# Autodesk Inventor assembly: Jersey_FEA_assembly
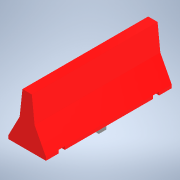
[picture p0: Inventor's stored thumbnail of the model, 180x180]
Saved by Autodesk Inventor 2022 (Build 260153000, 153)
## iProperties
Created: 2021-11-09
Part Number: Jersey_FEA_assembly
Document SubType Name: Assembly
Designer: kibandi
Author: kibandi
## Documents named in this file (3)
- C:\academics\YEAR 4\4.2\DOMS II\DOMS II projects\mechanical design\Jersey_FEA_assembly.iam
- C:\academics\YEAR 4\4.2\DOMS II\DOMS II projects\mechanical design\barrier_pneumatic_connector.ipt
- C:\academics\YEAR 4\4.2\DOMS II\DOMS II projects\mechanical design\Jersey Curb.ipt
## Components (2 placed, 2 different names)
1. barrier_pneumatic_connector:1 — Mate:2, Mate:4, Mate:7
2. Jersey Curb:1 — Mate:1, Mate:3, Mate:5, Mate:7
## Relationships (7: Mate 7)
- Mate:1: Jersey Curb:1
- Mate:2: barrier_pneumatic_connector:1
- Mate:3: Jersey Curb:1
- Mate:4: barrier_pneumatic_connector:1
- Mate:5: Jersey Curb:1
- Mate:6
- Mate:7: barrier_pneumatic_connector:1 ↔ Jersey Curb:1
